# Autodesk Inventor assembly: back wheel
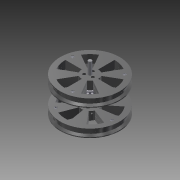
[picture p0: Inventor's stored thumbnail of the model, 180x180]
Saved by Autodesk Inventor 2011 (Build 150239000, 239)
## iProperties
Created: 2010-04-18
Part Number: back wheel
Document SubType Name: Assembly
Designer: lucio
Mass: 433.364 g
Surface Area: 1511.73 cm^2
Volume: 417.556 cm^3
Density: 1.03786 g/cm^3
Author: lucio
## Documents named in this file (4)
- C:\Users\lucio\Documents\Inventor\caterpillar\back wheel.iam
- C:\Users\lucio\Documents\Inventor\caterpillar\base wheel.iam
- C:\Users\lucio\Documents\Inventor\caterpillar\sprocket.ipt
- C:\Users\lucio\Documents\Inventor\caterpillar\back axle.ipt
## Components (4 placed, 3 different names)
1. back axle:1 — Mate:2, Flush:1, Mate:4, Mate:6
2. base wheel:1 [sub-assembly] — Mate:2, Flush:1, Mate:3
3. base wheel:2 [sub-assembly] — Mate:5, Mate:6
4. sprocket:1 — Mate:3, Mate:4, Mate:5
## Relationships (6: Mate 5, Flush 1)
- Mate:2: back axle:1 ↔ base wheel:1
- Flush:1 (12 mm): back axle:1 ↔ base wheel:1
- Mate:3 (32 mm): base wheel:1 ↔ sprocket:1
- Mate:4: back axle:1 ↔ sprocket:1
- Mate:5 (2 mm): base wheel:2 ↔ sprocket:1
- Mate:6: back axle:1 ↔ base wheel:2
